# Autodesk Inventor assembly: Motor_Assembly
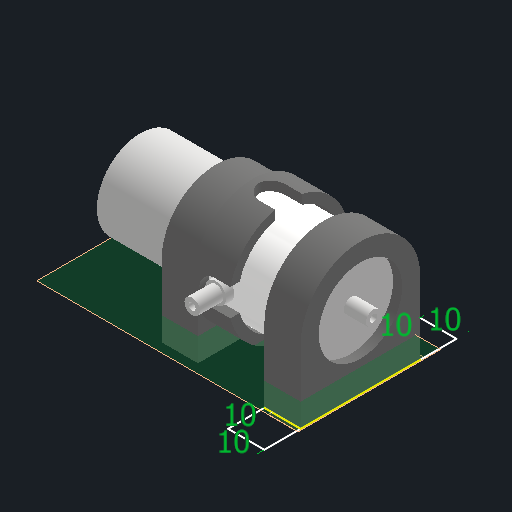
[picture p0: Inventor's stored thumbnail of the model, 512x512]
Saved by Autodesk Inventor 2026.2 (Build 302298000, 298)
## iProperties
Created: 2026-02-02
Part Number: Motor_Assembly
Document SubType Name: Assembly
Designer: vckot
Author: vckot
## Documents named in this file (4)
- C:\Users\vckot\OneDrive\Documents\Vaibhav\capstone\CAD_files\Motor\Motor_Assembly.iam
- C:\Users\vckot\OneDrive\Documents\Vaibhav\capstone\CAD_files\Motor\Adafruit_1528_4699_ND.ipt
- C:\Users\vckot\OneDrive\Documents\Vaibhav\capstone\CAD_files\Motor\Adafruit_1528_4699_ND_House_01.ipt
- C:\Users\vckot\OneDrive\Documents\Vaibhav\capstone\CAD_files\Motor\Adafruit_1528_4699_ND_House_02.ipt
## Components (3 placed, 3 different names)
1. Adafruit_1528_4699_ND:1 — Mate:1, Mate:3, Mate:4, Mate:5
2. Adafruit_1528_4699_ND_House_01:1 — Mate:1, Flush:1, Mate:5
3. Adafruit_1528_4699_ND_House_02:1 — Mate:3, Mate:4, Flush:1
## Relationships (5: Mate 4, Flush 1)
- Mate:1: Adafruit_1528_4699_ND:1 ↔ Adafruit_1528_4699_ND_House_01:1
- Mate:3: Adafruit_1528_4699_ND:1 ↔ Adafruit_1528_4699_ND_House_02:1
- Mate:4: Adafruit_1528_4699_ND:1 ↔ Adafruit_1528_4699_ND_House_02:1
- Flush:1: Adafruit_1528_4699_ND_House_01:1 ↔ Adafruit_1528_4699_ND_House_02:1
- Mate:5: Adafruit_1528_4699_ND:1 ↔ Adafruit_1528_4699_ND_House_01:1
